# Autodesk Inventor assembly: Assembly1
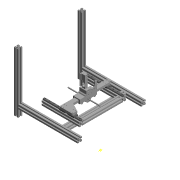
[picture p0: Inventor's stored thumbnail of the model, 180x180]
Saved by Autodesk Inventor 2016 (Build 200138000, 138)
## iProperties
Created: 2016-12-22
Part Number: Assembly1
Document SubType Name: Assembly
Designer: inorn
Author: inorn
## Documents named in this file (17)
- D:\Dropbox\KAIST\HCIL\Research\Switches\FD curve measure\Assembly1.iam
- D:\Dropbox\KAIST\HCIL\Research\Switches\FD curve measure\HorizontalBridge.ipt
- D:\Dropbox\Soruces\3d_Print\THK_RSR9KM1175750721000\AIS2016\RSR9KM3Slide.ipt
- D:\Dropbox\Soruces\3d_Print\THK_RSR9KM1175750721000\AIS2016\RSR9KM1757_51 Track.ipt
- D:\Dropbox\KAIST\HCIL\Research\Switches\FD curve measure\Profile.ipt
- D:\Dropbox\KAIST\HCIL\Research\Switches\FD curve measure\Profile_CPY.ipt
- D:\Dropbox\KAIST\HCIL\Research\Switches\FD curve measure\Profile_CPY1.ipt
- D:\Dropbox\KAIST\HCIL\Research\Switches\FD curve measure\NEMA17.ipt
- D:\Dropbox\KAIST\HCIL\Research\Switches\FD curve measure\motor_coupling.ipt
- D:\Dropbox\KAIST\HCIL\Research\Switches\FD curve measure\Screw.ipt
- D:\Dropbox\KAIST\HCIL\Research\Switches\FD curve measure\Nut.ipt
- D:\Dropbox\KAIST\HCIL\Research\Switches\FD curve measure\LoadCell.ipt
- D:\Dropbox\KAIST\HCIL\Research\Switches\FD curve measure\Profile_CPY2.ipt
- D:\Dropbox\KAIST\HCIL\Research\Switches\FD curve measure\Base.ipt
- D:\Dropbox\KAIST\HCIL\Research\Switches\Physical_button_simulator\Connector.ipt
- D:\Dropbox\KAIST\HCIL\Research\Switches\Physical_button_simulator\Connector_cap.ipt
- D:\Dropbox\KAIST\HCIL\Research\Switches\Physical_button_simulator\Scale_presser.ipt
## Components (23 placed, 16 different names)
1. HorizontalBridge:1 — Flush:1, Mate:1, Mate:2, Cylindrical:1, Cylindrical:2, Mate:13, Cylindrical:8, Cylindrical:9, Flush:17, Flush:19
2. RSR9KM3Slide:1 — Mate:1, Mate:4, Mate:5, Cylindrical:9
3. RSR9KM3Slide:2 — Mate:2, Cylindrical:1, Cylindrical:2, Mate:3, Mate:6
4. RSR9KM1757_51 Track:1 — Mate:3, Mate:6, Flush:2, Mate:7, Flush:3
5. RSR9KM1757_51 Track:2 — Mate:4, Mate:5, Flush:2, Mate:8, Flush:4, Mate:14, Mate:15
6. Profile:2 — Mate:7, Flush:3, Flush:5
7. Profile_CPY:1 — Mate:8, Flush:4, Flush:5, Mate:9, Flush:6, Flush:7, Mate:17, Flush:9
8. Profile_CPY1:1 — Mate:9, Flush:6, Flush:7, Mate:16, Flush:16, Mate:23, Mate:24
9. NEMA17:1 — Cylindrical:5, Mate:12, Flush:16, Mate:23, Mate:24
10. motor_coupling:1 — Cylindrical:5, Mate:11, Cylindrical:6, Mate:12
11. Screw:1 — Mate:11, Cylindrical:6, Rotational:1
12. LoadCell:1 — Mate:13, Flush:18, Mate:25, Flush:20
13. RSR9KM3Slide:3 — Mate:14, Mate:15, Cylindrical:8
14. Profile_CPY2:1 — Mate:16, Mate:17, Flush:9, Mate:18, Flush:10, Flush:11, Mate:19
15. Profile_CPY2:2 — Mate:18, Flush:10, Flush:12, Flush:14, Mate:21
16. Profile_CPY2:3 — Flush:11, Mate:19, Flush:12, Mate:20, Flush:13
17. Profile_CPY2:4 — Mate:20, Flush:13, Flush:15, Mate:22
18. Profile_CPY2:5 — Flush:14, Mate:21, Flush:15
19. Base:1 — Mate:22
20. Nut:1 — Rotational:1
21. Connector:1 — Flush:17, Flush:18, Mate:25
22. Connector_cap:1 — Flush:19
23. Scale_presser:1 — Flush:20
## Relationships (50: Mate 24, Flush 19, CylindricalJoint 6, RevoluteJoint 1)
- Flush:1: HorizontalBridge:1
- Mate:1: HorizontalBridge:1 ↔ RSR9KM3Slide:1
- Mate:2: HorizontalBridge:1 ↔ RSR9KM3Slide:2
- Cylindrical:1: HorizontalBridge:1 ↔ RSR9KM3Slide:2
- Cylindrical:2: HorizontalBridge:1 ↔ RSR9KM3Slide:2
- Mate:3: RSR9KM3Slide:2 ↔ RSR9KM1757_51 Track:1
- Mate:4: RSR9KM3Slide:1 ↔ RSR9KM1757_51 Track:2
- Mate:5: RSR9KM3Slide:1 ↔ RSR9KM1757_51 Track:2
- Mate:6: RSR9KM3Slide:2 ↔ RSR9KM1757_51 Track:1
- Flush:2: RSR9KM1757_51 Track:1 ↔ RSR9KM1757_51 Track:2
- Mate:7: RSR9KM1757_51 Track:1 ↔ Profile:2
- Flush:3 (-5.5 mm): RSR9KM1757_51 Track:1 ↔ Profile:2
- Mate:8: RSR9KM1757_51 Track:2 ↔ Profile_CPY:1
- Flush:4 (5.5 mm): RSR9KM1757_51 Track:2 ↔ Profile_CPY:1
- Flush:5: Profile:2 ↔ Profile_CPY:1
- Mate:9: Profile_CPY:1 ↔ Profile_CPY1:1
- Flush:6: Profile_CPY:1 ↔ Profile_CPY1:1
- Flush:7: Profile_CPY:1 ↔ Profile_CPY1:1
- Cylindrical:5: NEMA17:1 ↔ motor_coupling:1
- Mate:11 (-6 mm): motor_coupling:1 ↔ Screw:1
- Cylindrical:6: motor_coupling:1 ↔ Screw:1
- Mate:12 (14 mm): NEMA17:1 ↔ motor_coupling:1
- Mate:13: HorizontalBridge:1 ↔ LoadCell:1
- Mate:14: RSR9KM1757_51 Track:2 ↔ RSR9KM3Slide:3
- Mate:15: RSR9KM1757_51 Track:2 ↔ RSR9KM3Slide:3
- Cylindrical:8: HorizontalBridge:1 ↔ RSR9KM3Slide:3
- Cylindrical:9: HorizontalBridge:1 ↔ RSR9KM3Slide:1
- Mate:16 (-50 mm): Profile_CPY1:1 ↔ Profile_CPY2:1
- Mate:17: Profile_CPY:1 ↔ Profile_CPY2:1
- Flush:9 (-30 mm): Profile_CPY:1 ↔ Profile_CPY2:1
- Mate:18: Profile_CPY2:1 ↔ Profile_CPY2:2
- Flush:10: Profile_CPY2:1 ↔ Profile_CPY2:2
- Flush:11: Profile_CPY2:1 ↔ Profile_CPY2:3
- Mate:19: Profile_CPY2:1 ↔ Profile_CPY2:3
- Flush:12: Profile_CPY2:2 ↔ Profile_CPY2:3
- Mate:20: Profile_CPY2:3 ↔ Profile_CPY2:4
- Flush:13: Profile_CPY2:3 ↔ Profile_CPY2:4
- Flush:14: Profile_CPY2:2 ↔ Profile_CPY2:5
- Mate:21: Profile_CPY2:2 ↔ Profile_CPY2:5
- Flush:15: Profile_CPY2:4 ↔ Profile_CPY2:5
- Mate:22: Profile_CPY2:4 ↔ Base:1
- Flush:16 (67 mm): Profile_CPY1:1 ↔ NEMA17:1
- Mate:23 (6.3 mm): Profile_CPY1:1 ↔ NEMA17:1
- Mate:24 (19.08 mm): Profile_CPY1:1 ↔ NEMA17:1
- Rotational:1 [RevoluteJoint]: Screw:1 ↔ Nut:1
- Flush:17: HorizontalBridge:1 ↔ Connector:1
- Flush:18 (-5 mm): LoadCell:1 ↔ Connector:1
- Mate:25: LoadCell:1 ↔ Connector:1
- Flush:19: HorizontalBridge:1 ↔ Connector_cap:1
- Flush:20: LoadCell:1 ↔ Scale_presser:1
